# Autodesk Inventor assembly: Connect_Lower
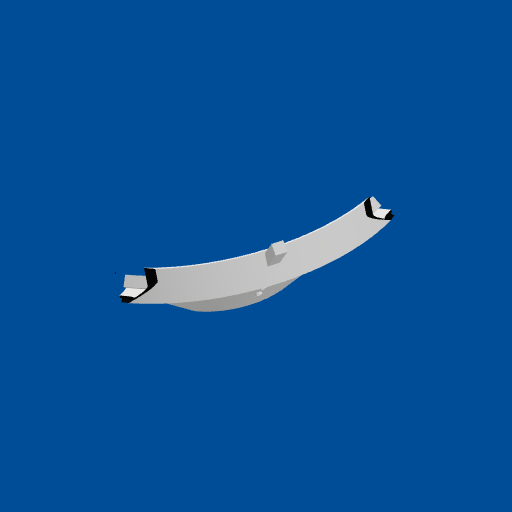
[picture p0: Inventor's stored thumbnail of the model, 512x512]
Saved by Autodesk Inventor 2026.2 (Build 302298000, 298)
## iProperties
Created: 2025-12-16
Part Number: Connect_Lower
Document SubType Name: Assembly
Designer: Thoma
Author: Thoma
## Documents named in this file (3)
- C:\Users\Thoma\OneDrive\Desktop\dir\telescope_cover\cover\Cover_Connect_Lower.iam
- C:\Users\Thoma\OneDrive\Desktop\dir\telescope_cover\cover\Cover_Lower_v2.ipt
- C:\Users\Thoma\OneDrive\Desktop\dir\telescope_cover\cover\rod.ipt
## Components (2 placed, 2 different names)
1. Cover_Lower_v2:1 — Flush:1, Flush:2
2. rod:1 — Flush:1, Flush:2
## Relationships (2: Flush 2)
- Flush:1: Cover_Lower_v2:1 ↔ rod:1
- Flush:2: Cover_Lower_v2:1 ↔ rod:1
